# Autodesk Inventor assembly: Robot
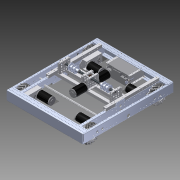
[picture p0: Inventor's stored thumbnail of the model, 180x180]
Saved by Autodesk Inventor 2015 SP1 (Build 190203100, 203)
## iProperties
Created: 2015-01-10
Part Number: Robot
Document SubType Name: Assembly
Designer: Jarod
Author: Jarod
## Documents named in this file (21)
- F:\Robotics\FRC\2015\CAD\Robot\Chassis\Chassis.iam
- F:\Robotics\FRC\2015\CAD\Robot\Chassis\Imported Components\AM14U2 End Sheet\AM14U2 End Sheet.ipt
- F:\Robotics\FRC\2015\CAD\Robot\Chassis\Imported Components\AM14U2 Inside Sheet\AM14U2 Inside Sheet.ipt
- F:\Robotics\FRC\2015\CAD\Robot\Chassis\Imported Components\AM14U2 Outside Sheet\AM14U2 Outside Sheet.ipt
- F:\Robotics\FRC\2015\CAD\Robot\Chassis\Imported Components\hub hex 0.5in\hub hex 0.5in.ipt
- F:\Robotics\FRC\2015\CAD\Robot\Chassis\Imported Components\Toughbox nano hex\Toughbox nano hex.iam
- F:\Robotics\FRC\2015\CAD\Robot\Chassis\ToughBox Nano Mounting Plate.ipt
- F:\Robotics\FRC\2015\CAD\Robot\Chassis\Imported Components\mecanum 6in left\mecanum 6in left.iam
- F:\Robotics\FRC\2015\CAD\Robot\Chassis\Imported Components\mecanum 6in right\mecanum 6in right.iam
- F:\Robotics\FRC\2015\CAD\Robot\Chassis\Imported Components\Battery Holder\Battery Holder.iam
- F:\Robotics\FRC\2015\CAD\Robot\Chassis\battery.ipt
- F:\Robotics\FRC\2015\CAD\Robot\Chassis\polycarb base.ipt
- F:\Robotics\FRC\2015\CAD\Robot\Chassis\churro.ipt
- F:\Robotics\FRC\2015\CAD\Robot\Chassis\churro long.ipt
- F:\Robotics\FRC\2015\CAD\Robot\Chassis\Imported Components\0.5 Hex Shaft Collar\0.5 Hex Shaft Collar.ipt
- F:\Robotics\FRC\2015\CAD\Robot\Chassis\mounting block lengthwise.ipt
- F:\Robotics\FRC\2015\CAD\Robot\Chassis\mounting block horizontal.ipt
- F:\Robotics\FRC\2015\CAD\Robot\Chassis\Imported Components\0.5 Hex Bearing\0.5 Hex Bearing.ipt
- F:\Robotics\FRC\2015\CAD\Robot\Chassis\0.5 hex shaft.ipt
- F:\Robotics\FRC\2015\CAD\Robot\Chassis\Imported Components\RAW gearbox\RAW gearbox.iam
- F:\Robotics\FRC\2015\CAD\Robot\Chassis\Imported Components\RAW gearbox\outside plate AB.ipt
## Components (53 placed, 20 different names)
1. AM14U2 End Sheet:1 — Mate:1, Flush:1, Flush:2, Mate:2, Mate:12, Mate:13, Mate:14, Mate:15, Mate:16, Mate:17, Mate:18, Mate:54, Mate:56, Mate:58, Mate:59, Mate:60, Mate:61, Mate:72, Mate:73
2. AM14U2 End Sheet:2 — Mate:19, Mate:20, Mate:21, Mate:55, Mate:57, Mate:66, Mate:67, Mate:68, Mate:70
3. AM14U2 Inside Sheet:1 — Mate:12, Mate:47, Mate:49, Flush:7, Flush:8, Mate:60, Mate:61, Mate:62, Mate:63, Flush:11, Mate:74, Mate:75, Mate:78, Mate:79, Mate:82, Mate:83, Mate:84, Mate:85, Mate:122, Mate:155, Mate:156
4. AM14U2 Inside Sheet:2 — Mate:2, Mate:46, Mate:48, Flush:9, Flush:10, Mate:58, Mate:59, Mate:64, Mate:65, Mate:76, Mate:77, Mate:80, Mate:81, Mate:125, Mate:157, Mate:158
5. AM14U2 Outside Sheet:1 — Mate:13, Mate:14, Mate:15, Mate:19, Mate:20, Mate:21
6. AM14U2 Outside Sheet:2 — Mate:16, Mate:17, Mate:18
7. mounting block lengthwise:1 — Mate:122, Mate:155, Mate:156, Mate:185, Mate:186, Mate:237, Mate:238
8. mounting block lengthwise:2 — Mate:125, Mate:157, Mate:158, Mate:239, Mate:240
9. mounting block horizontal:1 — Mate:185, Mate:236, Mate:237, Mate:240, Mate:242, Mate:244, Mate:245, Mate:246, Mate:247
10. mounting block horizontal:2 — Mate:186, Mate:238, Mate:239, Mate:241, Mate:243, Mate:248
11. churro:1 — Mate:74, Mate:79
12. churro:2 — Mate:75, Mate:78
13. churro:3 — Mate:76, Mate:81
14. churro:4 — Mate:77, Mate:80
15. churro long:1 — Mate:82, Mate:84
16. churro long:2 — Mate:83, Mate:85
17. Battery Holder:1 [sub-assembly] — Mate:66, Mate:67, Mate:68, Mate:69, Mate:71
18. battery:1 — Mate:69, Mate:70, Mate:71
19. polycarb base:1 — Mate:72, Flush:11, Mate:73
20. ToughBox Nano Mounting Plate:1 — Mate:38, Flush:3, Mate:39, Mate:47
21. ToughBox Nano Mounting Plate:2 — Mate:40, Flush:4, Mate:41, Mate:49
22. ToughBox Nano Mounting Plate:3 — Mate:44, Flush:6, Mate:45, Mate:46
23. ToughBox Nano Mounting Plate:4 — Mate:42, Flush:5, Mate:43, Mate:48
24. Toughbox nano hex:1 [sub-assembly] — Mate:23, Mate:25, Mate:38, Flush:3, Mate:39, Mate:54, Flush:7
25. Toughbox nano hex:2 [sub-assembly] — Mate:26, Mate:29, Mate:40, Flush:4, Mate:41, Mate:55, Flush:8
26. Toughbox nano hex:3 [sub-assembly] — Mate:30, Mate:33, Mate:44, Flush:6, Mate:45, Flush:9, Mate:56
27. Toughbox nano hex:4 [sub-assembly] — Mate:36, Mate:42, Flush:5, Mate:43, Mate:57, Flush:10
28. hub hex 0.5in:1 — Mate:23, Mate:24, Mate:63
29. hub hex 0.5in:2 — Mate:26, Mate:28, Mate:62
30. hub hex 0.5in:3 — Mate:30, Mate:32, Mate:64
31. hub hex 0.5in:4 — Mate:34, Mate:35, Mate:36, Mate:65
32. mecanum 6in left:1 [sub-assembly] — Mate:24, Mate:25
33. mecanum 6in left:2 [sub-assembly] — Mate:34, Mate:35
34. mecanum 6in right:1 [sub-assembly] — Mate:28, Mate:29
35. mecanum 6in right:2 [sub-assembly] — Mate:32, Mate:33
36. RAW gearbox:1 [sub-assembly] — Mate:236, Mate:241, Mate:242
37. outside plate AB:1 — Mate:243, Mate:244, Mate:245, Mate:360, Mate:361
38. outside plate AB:2 — Mate:246, Mate:247, Mate:248, Mate:356, Mate:357
39. 0.5 hex shaft:1 — Mate:365, Mate:366, Flush:12
40. 0.5 Hex Bearing:1 — Mate:360, Mate:361, Mate:362, Mate:363, Mate:364, Mate:369, Mate:371, Mate:373, Mate:380
41. 0.5 Hex Bearing:2 — Mate:356, Mate:357, Mate:358, Mate:365, Mate:366, Mate:375, Mate:377, Mate:379, Flush:12, Mate:381, Mate:382, Mate:383
42. hub hex 0.5in:5 — Mate:364, Mate:368, Mate:387
43. hub hex 0.5in:6 — Mate:368, Mate:369, Mate:370
44. hub hex 0.5in:7 — Mate:370, Mate:371, Mate:386
45. hub hex 0.5in:8 — Mate:378, Mate:379, Mate:385
46. hub hex 0.5in:9 — Mate:376, Mate:377, Mate:378
47. hub hex 0.5in:10 — Mate:375, Mate:376, Mate:384
48. 0.5 Hex Shaft Collar:2 — Mate:362, Mate:363, Mate:388
49. 0.5 Hex Shaft Collar:3 — Mate:373, Mate:387, Mate:388
50. 0.5 Hex Shaft Collar:4 — Mate:380, Mate:386
51. 0.5 Hex Shaft Collar:5 — Mate:358, Mate:385
52. 0.5 Hex Shaft Collar:7 — Mate:382, Mate:383, Mate:389
53. 0.5 Hex Shaft Collar:6 — Mate:381, Mate:384, Mate:389
## Relationships (131: Mate 119, Flush 12)
- Mate:1: AM14U2 End Sheet:1
- Flush:1: AM14U2 End Sheet:1
- Flush:2: AM14U2 End Sheet:1
- Mate:2: AM14U2 End Sheet:1 ↔ AM14U2 Inside Sheet:2
- Mate:12: AM14U2 End Sheet:1 ↔ AM14U2 Inside Sheet:1
- Mate:13: AM14U2 End Sheet:1 ↔ AM14U2 Outside Sheet:1
- Mate:14: AM14U2 End Sheet:1 ↔ AM14U2 Outside Sheet:1
- Mate:15: AM14U2 End Sheet:1 ↔ AM14U2 Outside Sheet:1
- Mate:16: AM14U2 End Sheet:1 ↔ AM14U2 Outside Sheet:2
- Mate:17: AM14U2 End Sheet:1 ↔ AM14U2 Outside Sheet:2
- Mate:18: AM14U2 End Sheet:1 ↔ AM14U2 Outside Sheet:2
- Mate:19: AM14U2 End Sheet:2 ↔ AM14U2 Outside Sheet:1
- Mate:20: AM14U2 End Sheet:2 ↔ AM14U2 Outside Sheet:1
- Mate:21: AM14U2 End Sheet:2 ↔ AM14U2 Outside Sheet:1
- Mate:23: Toughbox nano hex:1 ↔ hub hex 0.5in:1
- Mate:24: hub hex 0.5in:1 ↔ mecanum 6in left:1
- Mate:25: Toughbox nano hex:1 ↔ mecanum 6in left:1
- Mate:26: Toughbox nano hex:2 ↔ hub hex 0.5in:2
- Mate:28: hub hex 0.5in:2 ↔ mecanum 6in right:1
- Mate:29: Toughbox nano hex:2 ↔ mecanum 6in right:1
- Mate:30: Toughbox nano hex:3 ↔ hub hex 0.5in:3
- Mate:32: hub hex 0.5in:3 ↔ mecanum 6in right:2
- Mate:33: Toughbox nano hex:3 ↔ mecanum 6in right:2
- Mate:34: hub hex 0.5in:4 ↔ mecanum 6in left:2
- Mate:35: hub hex 0.5in:4 ↔ mecanum 6in left:2
- Mate:36: Toughbox nano hex:4 ↔ hub hex 0.5in:4
- Mate:38: ToughBox Nano Mounting Plate:1 ↔ Toughbox nano hex:1
- Flush:3: ToughBox Nano Mounting Plate:1 ↔ Toughbox nano hex:1
- Mate:39: ToughBox Nano Mounting Plate:1 ↔ Toughbox nano hex:1
- Mate:40: ToughBox Nano Mounting Plate:2 ↔ Toughbox nano hex:2
- Flush:4: ToughBox Nano Mounting Plate:2 ↔ Toughbox nano hex:2
- Mate:41: ToughBox Nano Mounting Plate:2 ↔ Toughbox nano hex:2
- Mate:42: ToughBox Nano Mounting Plate:4 ↔ Toughbox nano hex:4
- Flush:5: ToughBox Nano Mounting Plate:4 ↔ Toughbox nano hex:4
- Mate:43: ToughBox Nano Mounting Plate:4 ↔ Toughbox nano hex:4
- Mate:44: ToughBox Nano Mounting Plate:3 ↔ Toughbox nano hex:3
- Flush:6: ToughBox Nano Mounting Plate:3 ↔ Toughbox nano hex:3
- Mate:45: ToughBox Nano Mounting Plate:3 ↔ Toughbox nano hex:3
- Mate:46: AM14U2 Inside Sheet:2 ↔ ToughBox Nano Mounting Plate:3
- Mate:47: AM14U2 Inside Sheet:1 ↔ ToughBox Nano Mounting Plate:1
- Mate:48: AM14U2 Inside Sheet:2 ↔ ToughBox Nano Mounting Plate:4
- Mate:49: AM14U2 Inside Sheet:1 ↔ ToughBox Nano Mounting Plate:2
- Mate:54 (64.6176 mm): AM14U2 End Sheet:1 ↔ Toughbox nano hex:1
- Flush:7 (-24.4856 mm): AM14U2 Inside Sheet:1 ↔ Toughbox nano hex:1
- Mate:55 (64.6176 mm): AM14U2 End Sheet:2 ↔ Toughbox nano hex:2
- Flush:8 (-24.4856 mm): AM14U2 Inside Sheet:1 ↔ Toughbox nano hex:2
- Flush:9 (-24.4856 mm): AM14U2 Inside Sheet:2 ↔ Toughbox nano hex:3
- Mate:56 (64.6176 mm): AM14U2 End Sheet:1 ↔ Toughbox nano hex:3
- Mate:57 (64.6176 mm): AM14U2 End Sheet:2 ↔ Toughbox nano hex:4
- Flush:10 (-24.4856 mm): AM14U2 Inside Sheet:2 ↔ Toughbox nano hex:4
- Mate:58: AM14U2 End Sheet:1 ↔ AM14U2 Inside Sheet:2
- Mate:59: AM14U2 End Sheet:1 ↔ AM14U2 Inside Sheet:2
- Mate:60: AM14U2 End Sheet:1 ↔ AM14U2 Inside Sheet:1
- Mate:61: AM14U2 End Sheet:1 ↔ AM14U2 Inside Sheet:1
- Mate:62: AM14U2 Inside Sheet:1 ↔ hub hex 0.5in:2
- Mate:63: AM14U2 Inside Sheet:1 ↔ hub hex 0.5in:1
- Mate:64: AM14U2 Inside Sheet:2 ↔ hub hex 0.5in:3
- Mate:65: AM14U2 Inside Sheet:2 ↔ hub hex 0.5in:4
- Mate:66: AM14U2 End Sheet:2 ↔ Battery Holder:1
- Mate:67: AM14U2 End Sheet:2 ↔ Battery Holder:1
- Mate:68: AM14U2 End Sheet:2 ↔ Battery Holder:1
- Mate:69: Battery Holder:1 ↔ battery:1
- Mate:70: AM14U2 End Sheet:2 ↔ battery:1
- Mate:71: Battery Holder:1 ↔ battery:1
- Mate:72: AM14U2 End Sheet:1 ↔ polycarb base:1
- Flush:11: AM14U2 Inside Sheet:1 ↔ polycarb base:1
- Mate:73: AM14U2 End Sheet:1 ↔ polycarb base:1
- Mate:74: AM14U2 Inside Sheet:1 ↔ churro:1
- Mate:75: AM14U2 Inside Sheet:1 ↔ churro:2
- Mate:76: AM14U2 Inside Sheet:2 ↔ churro:3
- Mate:77: AM14U2 Inside Sheet:2 ↔ churro:4
- Mate:78: AM14U2 Inside Sheet:1 ↔ churro:2
- Mate:79: AM14U2 Inside Sheet:1 ↔ churro:1
- Mate:80: AM14U2 Inside Sheet:2 ↔ churro:4
- Mate:81: AM14U2 Inside Sheet:2 ↔ churro:3
- Mate:82: AM14U2 Inside Sheet:1 ↔ churro long:1
- Mate:83: AM14U2 Inside Sheet:1 ↔ churro long:2
- Mate:84: AM14U2 Inside Sheet:1 ↔ churro long:1
- Mate:85: AM14U2 Inside Sheet:1 ↔ churro long:2
- Mate:122: AM14U2 Inside Sheet:1 ↔ mounting block lengthwise:1
- Mate:125: AM14U2 Inside Sheet:2 ↔ mounting block lengthwise:2
- Mate:155: AM14U2 Inside Sheet:1 ↔ mounting block lengthwise:1
- Mate:156: AM14U2 Inside Sheet:1 ↔ mounting block lengthwise:1
- Mate:157: AM14U2 Inside Sheet:2 ↔ mounting block lengthwise:2
- Mate:158: AM14U2 Inside Sheet:2 ↔ mounting block lengthwise:2
- Mate:185: mounting block lengthwise:1 ↔ mounting block horizontal:1
- Mate:186: mounting block lengthwise:1 ↔ mounting block horizontal:2
- Mate:236: mounting block horizontal:1 ↔ RAW gearbox:1
- Mate:237: mounting block lengthwise:1 ↔ mounting block horizontal:1
- Mate:238: mounting block lengthwise:1 ↔ mounting block horizontal:2
- Mate:239: mounting block lengthwise:2 ↔ mounting block horizontal:2
- Mate:240: mounting block lengthwise:2 ↔ mounting block horizontal:1
- Mate:241: mounting block horizontal:2 ↔ RAW gearbox:1
- Mate:242: mounting block horizontal:1 ↔ RAW gearbox:1
- Mate:243: mounting block horizontal:2 ↔ outside plate AB:1
- Mate:244: mounting block horizontal:1 ↔ outside plate AB:1
- Mate:245: mounting block horizontal:1 ↔ outside plate AB:1
- Mate:246: mounting block horizontal:1 ↔ outside plate AB:2
- Mate:247: mounting block horizontal:1 ↔ outside plate AB:2
- Mate:248: mounting block horizontal:2 ↔ outside plate AB:2
- Mate:356: outside plate AB:2 ↔ 0.5 Hex Bearing:2
- Mate:357: outside plate AB:2 ↔ 0.5 Hex Bearing:2
- Mate:358: 0.5 Hex Bearing:2 ↔ 0.5 Hex Shaft Collar:5
- Mate:360: outside plate AB:1 ↔ 0.5 Hex Bearing:1
- Mate:361: outside plate AB:1 ↔ 0.5 Hex Bearing:1
- Mate:362: 0.5 Hex Bearing:1 ↔ 0.5 Hex Shaft Collar:2
- Mate:363: 0.5 Hex Bearing:1 ↔ 0.5 Hex Shaft Collar:2
- Mate:364: 0.5 Hex Bearing:1 ↔ hub hex 0.5in:5
- Mate:365: 0.5 hex shaft:1 ↔ 0.5 Hex Bearing:2
- Mate:366: 0.5 hex shaft:1 ↔ 0.5 Hex Bearing:2
- Mate:368: hub hex 0.5in:5 ↔ hub hex 0.5in:6
- Mate:369: 0.5 Hex Bearing:1 ↔ hub hex 0.5in:6
- Mate:370: hub hex 0.5in:6 ↔ hub hex 0.5in:7
- Mate:371: 0.5 Hex Bearing:1 ↔ hub hex 0.5in:7
- Mate:373: 0.5 Hex Bearing:1 ↔ 0.5 Hex Shaft Collar:3
- Mate:375: 0.5 Hex Bearing:2 ↔ hub hex 0.5in:10
- Mate:376: hub hex 0.5in:9 ↔ hub hex 0.5in:10
- Mate:377: 0.5 Hex Bearing:2 ↔ hub hex 0.5in:9
- Mate:378: hub hex 0.5in:8 ↔ hub hex 0.5in:9
- Mate:379: 0.5 Hex Bearing:2 ↔ hub hex 0.5in:8
- Flush:12: 0.5 hex shaft:1 ↔ 0.5 Hex Bearing:2
- Mate:380: 0.5 Hex Bearing:1 ↔ 0.5 Hex Shaft Collar:4
- Mate:381: 0.5 Hex Bearing:2 ↔ 0.5 Hex Shaft Collar:6
- Mate:382: 0.5 Hex Bearing:2 ↔ 0.5 Hex Shaft Collar:7
- Mate:383: 0.5 Hex Bearing:2 ↔ 0.5 Hex Shaft Collar:7
- Mate:384: hub hex 0.5in:10 ↔ 0.5 Hex Shaft Collar:6
- Mate:385: hub hex 0.5in:8 ↔ 0.5 Hex Shaft Collar:5
- Mate:386: hub hex 0.5in:7 ↔ 0.5 Hex Shaft Collar:4
- Mate:387: hub hex 0.5in:5 ↔ 0.5 Hex Shaft Collar:3
- Mate:388 (31.75 mm): 0.5 Hex Shaft Collar:2 ↔ 0.5 Hex Shaft Collar:3
- Mate:389 (31.75 mm): 0.5 Hex Shaft Collar:7 ↔ 0.5 Hex Shaft Collar:6
